# Autodesk Inventor assembly: Final AssemblyV5
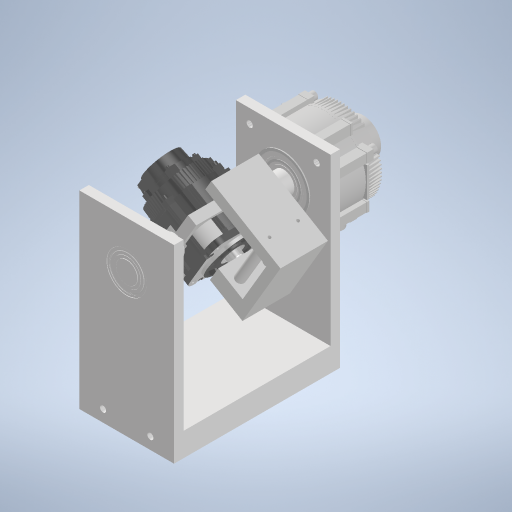
[picture p0: Inventor's stored thumbnail of the model, 512x512]
Saved by Autodesk Inventor 2024 (Build 280153000, 153)
## iProperties
Created: 2024-02-08
Part Number: Final AssemblyV5
Document SubType Name: Assembly
Designer: yusuf
Author: yusuf
## Documents named in this file (9)
- C:\Users\yusuf\Documents\DodgeBot\design\hardware\CAD_FILES\Final AssemblyV5.iam
- C:\Users\yusuf\Documents\DodgeBot\design\hardware\CAD_FILES\YASKAWA_USA_SGM7G30A6A61\AIS2024\SGM7G-30A6A61.iam
- C:\Users\yusuf\Documents\DodgeBot\design\hardware\CAD_FILES\FrontPlateV2.ipt
- C:\Users\yusuf\Documents\DodgeBot\design\hardware\CAD_FILES\SGM7G_20AxA61\SGM7G-20xxA61\ProE\SGM7G-20__a61_ProE\ProE\sgm7g_20__a61\sgm7g_20__a61.iam
- C:\Users\yusuf\Documents\DodgeBot\design\hardware\CAD_FILES\145100992-9-skf_bearing_6209-2z_2\skf_bearing_6209-2z_2.iam
- C:\Users\yusuf\Documents\DodgeBot\design\hardware\CAD_FILES\FloorMount.ipt
- C:\Users\yusuf\Documents\DodgeBot\design\hardware\CAD_FILES\FloorMountFacePlate.ipt
- C:\Users\yusuf\Documents\DodgeBot\design\hardware\CAD_FILES\EndEffectorMotorAdapter.ipt
- C:\Users\yusuf\Documents\DodgeBot\design\hardware\CAD_FILES\SupportRods.ipt
## Components (10 placed, 8 different names)
1. SGM7G-30A6A61:1 [sub-assembly] — Rigid:2
2. FrontPlateV2:1 — Rigid:1, Rotational:1
3. sgm7g_20__a61:1 [sub-assembly] — Rigid:1, Rotational:4
4. skf_bearing_6209-2z_2:1 [sub-assembly] — Rotational:3
5. skf_bearing_6209-2z_2:2 [sub-assembly] — Rotational:1, Rotational:2
6. FloorMount:1 — Rotational:2, Rigid:2, Rigid:3
7. FloorMountFacePlate:1 — Rigid:3, Rotational:3
8. EndEffectorMotorAdapter:1 — Rotational:4, Rigid:4, Rigid:5
9. SupportRods:1 — Rigid:5
10. SupportRods:2 — Rigid:4
## Relationships (9: WeldJoint 5, RevoluteJoint 4)
- Rigid:1 [WeldJoint] (-109 mm): FrontPlateV2:1 ↔ sgm7g_20__a61:1
- Rotational:1 [RevoluteJoint] (-49 mm): FrontPlateV2:1 ↔ skf_bearing_6209-2z_2:2
- Rotational:2 [RevoluteJoint]: skf_bearing_6209-2z_2:2 ↔ FloorMount:1
- Rigid:2 [WeldJoint]: SGM7G-30A6A61:1 ↔ FloorMount:1
- Rigid:3 [WeldJoint]: FloorMount:1 ↔ FloorMountFacePlate:1
- Rotational:3 [RevoluteJoint]: skf_bearing_6209-2z_2:1 ↔ FloorMountFacePlate:1
- Rotational:4 [RevoluteJoint]: sgm7g_20__a61:1 ↔ EndEffectorMotorAdapter:1
- Rigid:4 [WeldJoint]: EndEffectorMotorAdapter:1 ↔ SupportRods:2
- Rigid:5 [WeldJoint]: EndEffectorMotorAdapter:1 ↔ SupportRods:1
